# Autodesk Inventor assembly: Trunk
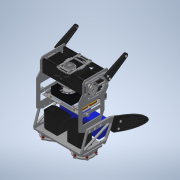
[picture p0: Inventor's stored thumbnail of the model, 180x180]
Saved by Autodesk Inventor 2020.4 (Build 244396000, 396)
## iProperties
Created: 2021-09-10
Part Number: Trunk
Document SubType Name: Assembly
Designer: Masato
Mass: 1616.91 g
Surface Area: 5782.28 cm^2
Volume: 882.028 cm^3
Density: 1.83317 g/cm^3
Author: Masato
## Documents named in this file (27)
- C:\Users\Masato\Documents\Inventor\CIT Brains_Inventor\OpenPlatform_ver3_0 - ve4_1 branch\UpperBody\Trunk\Trunk.iam
- C:\Users\Masato\Documents\Inventor\CIT Brains_Inventor\OpenPlatform_ver3_0 - ve4_1 branch\UpperBody\Trunk\Trunk_chest_horizontal_frame.ipt
- C:\Users\Masato\Documents\Inventor\CIT Brains_Inventor\OpenPlatform_ver3_0 - ve4_1 branch\UpperBody\Trunk\Trunk_chest_back_forth_frame.ipt
- C:\Users\Masato\Documents\Inventor\CIT Brains_Inventor\OpenPlatform_ver3_0 - ve4_1 branch\UpperBody\Trunk\Trunk_upper_flank_frame.ipt
- C:\Users\Masato\Documents\Inventor\CIT Brains_Inventor\OpenPlatform_ver3_0 - ve4_1 branch\UpperBody\Trunk\Trunk_shoulder_frame.ipt
- C:\Users\Masato\Documents\Inventor\CIT Brains_Inventor\OpenPlatform_ver3_0 - ve4_1 branch\UpperBody\Trunk\Trunk_handle_frame.ipt
- C:\Users\Masato\Documents\Inventor\CIT Brains_Inventor\OpenPlatform_ver3_0 - ve4_1 branch\Ready_Made\B3M11xx.ipt
- C:\Users\Masato\Documents\Inventor\CIT Brains_Inventor\OpenPlatform_ver3_0 - ve4_1 branch\Ready_Made\B3M10xx.ipt
- C:\Users\Masato\Documents\Inventor\CIT Brains_Inventor\OpenPlatform_ver3_0 - ve4_1 branch\UpperBody\Trunk\Trunk_shoulder_frame_MIR.ipt
- C:\Users\Masato\Documents\Inventor\CIT Brains_Inventor\OpenPlatform_ver3_0 - ve4_1 branch\UpperBody\Trunk\Trunk_lower_flank_frame.ipt
- C:\Users\Masato\Documents\Inventor\CIT Brains_Inventor\OpenPlatform_ver3_0 - ve4_1 branch\Ready_Made\Screw\SPNFL-BRN-M3-6.ipt
- C:\Users\Masato\Documents\Inventor\CIT Brains_Inventor\OpenPlatform_ver3_0 - ve4_1 branch\Ready_Made\Screw\M2_6-15.ipt
- C:\Users\Masato\Documents\Inventor\CIT Brains_Inventor\OpenPlatform_ver3_0 - ve4_1 branch\Ready_Made\Screw\M3-8.ipt
- C:\Users\Masato\Documents\Inventor\CIT Brains_Inventor\OpenPlatform_ver3_0 - ve4_1 branch\Ready_Made\Screw\M3-6.ipt
- C:\Users\Masato\Documents\Inventor\CIT Brains_Inventor\OpenPlatform_ver3_0 - ve4_1 branch\Ready_Made\Screw\M2_6-20.ipt
- C:\Users\Masato\Documents\Inventor\CIT Brains_Inventor\OpenPlatform_ver3_0 - ve4_1 branch\Ready_Made\BRU-309S.ipt
- C:\Users\Masato\Documents\Inventor\CIT Brains_Inventor\OpenPlatform_ver3_0 - ve4_1 branch\Ready_Made\UUW-0312-10BH.ipt
- C:\Users\Masato\Documents\Inventor\CIT Brains_Inventor\OpenPlatform_ver3_0 - ve4_1 branch\Ready_Made\ARU-306S.ipt
- C:\Users\Masato\Documents\Inventor\CIT Brains_Inventor\OpenPlatform_ver3_0 - ve4_1 branch\Ready_Made\SF319.ipt
- C:\Users\Masato\Documents\Inventor\CIT Brains_Inventor\OpenPlatform_ver3_0 - ve4_1 branch\UpperBody\Trunk\Trunk_back_bumper.ipt
- C:\Users\Masato\Documents\Inventor\CIT Brains_Inventor\OpenPlatform_ver3_0 - ve4_1 branch\Ready_Made\Screw\ClampHorn_Screw.ipt
- C:\Users\Masato\Documents\Inventor\CIT Brains_Inventor\OpenPlatform_ver3_0 - ve4_1 branch\Ready_Made\ClampHorn.ipt
- C:\Users\Masato\Documents\Inventor\CIT Brains_Inventor\OpenPlatform_ver3_0 - ve4_1 branch\Ready_Made\Jetson_Xavier_NX_DevKit_without_Wi-FiAntennas\Jetson_Xavier_NX_DevKit.ipt
- C:\Users\Masato\Documents\Inventor\CIT Brains_Inventor\OpenPlatform_ver3_0 - ve4_1 branch\Ready_Made\HP-G570-2600S3.ipt
- C:\Users\Masato\Documents\Inventor\CIT Brains_Inventor\OpenPlatform_ver3_0 - ve4_1 branch\UpperBody\Trunk\Trunk_lower_waisit_frame_.ipt
- C:\Users\Masato\Documents\Inventor\CIT Brains_Inventor\OpenPlatform_ver3_0 - ve4_1 branch\UpperBody\Trunk\CrossRollerBearing\BearingUnit.iam
- ClampHorn.ipt
## Components (98 placed, 25 different names)
1. Trunk_chest_horizontal_frame:1 — 挿入:172, 挿入:173, 挿入:174, 挿入:175, 挿入:177, 挿入:179, 挿入:255, 挿入:256, 挿入:261, 挿入:262, 挿入:347, 挿入:348
2. Trunk_chest_horizontal_frame:2 — 挿入:181, 挿入:182, 挿入:184, 挿入:185, 挿入:186, 挿入:187, 挿入:257, 挿入:258, 挿入:337, 挿入:338, 挿入:465, 挿入:466, 挿入:664, 挿入:665
3. Trunk_chest_back_forth_frame:1 — 挿入:115, 挿入:116, 挿入:117, 挿入:118, 挿入:172, 挿入:173, 挿入:181, 挿入:182
4. Trunk_chest_back_forth_frame:2 — 挿入:154, 挿入:155, 挿入:156, 挿入:157, 挿入:174, 挿入:175, 挿入:185, 挿入:187
5. Trunk_lower_flank_frame:1 — 挿入:501, 挿入:502, 挿入:668, 挿入:669, 挿入:692, 角度:3
6. Trunk_lower_flank_frame:2 — 挿入:499, 挿入:500, 挿入:666, 挿入:667, 挿入:691, メイト:3, メイト:4, 角度:2
7. Trunk_upper_flank_frame:1 — 挿入:115, 挿入:116, 挿入:156, 挿入:157, 挿入:226, 挿入:251, 挿入:252, 挿入:349, 挿入:350, フラッシュ:2, メイト:4, 挿入:699, 挿入:700, メイト:3
8. Trunk_upper_flank_frame:2 — 挿入:117, 挿入:118, 挿入:154, 挿入:155, 挿入:227, 挿入:253, 挿入:254, 挿入:351, 挿入:352, 挿入:697, 挿入:698
9. Trunk_shoulder_frame:1 — 挿入:559, 挿入:560, 挿入:561, 挿入:562, 挿入:563, 挿入:564, 挿入:565, 挿入:566, 挿入:571, 挿入:572, 挿入:573, 挿入:574, 挿入:699, 挿入:700
10. Trunk_shoulder_frame_MIR:1 — 挿入:581, 挿入:582, 挿入:583, 挿入:584, 挿入:587, 挿入:588, 挿入:589, 挿入:590, 挿入:591, 挿入:592, 挿入:593, 挿入:594, 挿入:595, 挿入:596, 挿入:697, 挿入:698
11. Trunk_handle_frame:1 — 挿入:263, 挿入:264, 挿入:267, 挿入:575, 挿入:576
12. Trunk_handle_frame:2 — 挿入:265, 挿入:266, 挿入:268, 挿入:597, 挿入:598
13. B3M11xx:3 — 挿入:177, 挿入:179, 挿入:184, 挿入:186, 挿入:681, 挿入:686
14. B3M10xx:4 — 挿入:559, 挿入:560, 挿入:561, 挿入:562, 挿入:679, 挿入:684
15. B3M10xx:5 — 挿入:581, 挿入:582, 挿入:583, 挿入:584, 挿入:680, 挿入:685
16. SPNFL-BRN-M3-6:1 — 挿入:226
17. SPNFL-BRN-M3-6:2 — 挿入:227
18. M3-6:1 — 挿入:251
19. M3-6:2 — 挿入:252
20. M3-6:3 — 挿入:254
21. M3-6:4 — 挿入:253
22. M3-6:5 — 挿入:256
23. M3-6:6 — 挿入:255
24. M3-6:7 — 挿入:258
25. M3-6:8 — 挿入:257
26. M2_6-15:11 — 挿入:261
27. M2_6-15:12 — 挿入:262
28. M3-6:9 — 挿入:263
29. M3-6:10 — 挿入:264
30. M3-6:11 — 挿入:266
31. M3-6:12 — 挿入:265
32. M3-8:11 — 挿入:267
33. M3-8:12 — 挿入:268
34. M2_6-15:13 — 挿入:564
35. M2_6-15:14 — 挿入:563
36. M2_6-15:15 — 挿入:566
37. M2_6-15:16 — 挿入:565
38. M2_6-15:17 — 挿入:591
39. M2_6-15:18 — 挿入:592
40. M2_6-15:19 — 挿入:589
41. M2_6-15:20 — 挿入:590
42. M3-6:19 — 挿入:587
43. M3-6:20 — 挿入:588
44. M2_6-20:9 — 挿入:465
45. M2_6-20:10 — 挿入:466
46. M2_6-20:11 — 挿入:337
47. M2_6-20:12 — 挿入:338
48. M3-6:29 — 挿入:347
49. M3-6:30 — 挿入:348
50. M3-6:31 — 挿入:349
51. M3-6:32 — 挿入:350
52. M3-6:33 — 挿入:351
53. M3-6:34 — 挿入:352
54. BRU-309S:9 — 挿入:497, 挿入:503
55. BRU-309S:10 — 挿入:498, 挿入:504
56. BRU-309S:11 — 挿入:496, 挿入:506
57. BRU-309S:12 — 挿入:495, 挿入:505
58. UUW-0312-10BH:1 — 挿入:495, 挿入:507
59. UUW-0312-10BH:2 — 挿入:496, 挿入:508
60. UUW-0312-10BH:3 — 挿入:497, 挿入:509
61. UUW-0312-10BH:4 — 挿入:498, 挿入:510
62. UUW-0312-10BH:5 — 挿入:499, 挿入:505, 挿入:672
63. UUW-0312-10BH:6 — 挿入:500, 挿入:506, 挿入:673
64. UUW-0312-10BH:7 — 挿入:501, 挿入:503, 挿入:674
65. UUW-0312-10BH:8 — 挿入:502, 挿入:504, 挿入:675
66. M3-6:43 — 挿入:507
67. M3-6:44 — 挿入:508
68. M3-6:45 — 挿入:510
69. M3-6:46 — 挿入:509
70. ARU-306S:1 — 挿入:571, 挿入:576
71. ARU-306S:2 — 挿入:572, 挿入:575
72. M3-6:55 — 挿入:573
73. M3-6:56 — 挿入:574
74. M3-6:57 — 挿入:593
75. M3-6:58 — 挿入:594
76. ARU-306S:3 — 挿入:595, 挿入:597
77. ARU-306S:4 — 挿入:596, 挿入:598
78. M3-6:59 — 挿入:664
79. M3-6:60 — 挿入:665
80. SF319:1 — 挿入:666
81. SF319:2 — 挿入:667
82. SF319:3 — 挿入:668
83. SF319:4 — 挿入:669
84. Trunk_back_bumper:1 — 挿入:672, 挿入:673
85. Trunk_back_bumper:2 — 挿入:674, 挿入:675
86. ClampHorn_Screw:3 — 挿入:684
87. ClampHorn_Screw:4 — 挿入:685
88. ClampHorn_Screw:5 — 挿入:686
89. ClampHorn:3 — 挿入:679
90. ClampHorn:4 — 挿入:680
91. ClampHorn:5 — 挿入:681
92. B3M11xx:1 — 挿入:689, 挿入:690
93. B3M11xx:2 — 挿入:687, 挿入:688
94. Jetson_Xavier_NX_DevKit:1
95. HP-G570-2600S3:1
96. Trunk_lower_waisit_frame_:1 — フラッシュ:1, 挿入:687, 挿入:688, 挿入:689, 挿入:690, 挿入:691, 挿入:692, フラッシュ:2, 角度:2, 角度:3, 挿入:693, 挿入:694, 挿入:695, 挿入:696, メイト:5
97. BearingUnit:1 [sub-assembly] — 挿入:694, 挿入:695
98. BearingUnit:2 [sub-assembly] — 挿入:693, 挿入:696
## Relationships (131: Insert 124, Mate 3, Flush 2, Angle 2)
- 挿入:115 [Insert]: Trunk_chest_back_forth_frame:1 ↔ Trunk_upper_flank_frame:1
- 挿入:116 [Insert]: Trunk_chest_back_forth_frame:1 ↔ Trunk_upper_flank_frame:1
- 挿入:117 [Insert]: Trunk_chest_back_forth_frame:1 ↔ Trunk_upper_flank_frame:2
- 挿入:118 [Insert]: Trunk_chest_back_forth_frame:1 ↔ Trunk_upper_flank_frame:2
- 挿入:154 [Insert]: Trunk_chest_back_forth_frame:2 ↔ Trunk_upper_flank_frame:2
- 挿入:155 [Insert]: Trunk_chest_back_forth_frame:2 ↔ Trunk_upper_flank_frame:2
- 挿入:156 [Insert]: Trunk_chest_back_forth_frame:2 ↔ Trunk_upper_flank_frame:1
- 挿入:157 [Insert]: Trunk_chest_back_forth_frame:2 ↔ Trunk_upper_flank_frame:1
- 挿入:172 [Insert]: Trunk_chest_horizontal_frame:1 ↔ Trunk_chest_back_forth_frame:1
- 挿入:173 [Insert]: Trunk_chest_horizontal_frame:1 ↔ Trunk_chest_back_forth_frame:1
- 挿入:174 [Insert]: Trunk_chest_horizontal_frame:1 ↔ Trunk_chest_back_forth_frame:2
- 挿入:175 [Insert]: Trunk_chest_horizontal_frame:1 ↔ Trunk_chest_back_forth_frame:2
- 挿入:177 [Insert]: Trunk_chest_horizontal_frame:1 ↔ B3M11xx:3
- 挿入:179 [Insert]: Trunk_chest_horizontal_frame:1 ↔ B3M11xx:3
- 挿入:181 [Insert]: Trunk_chest_horizontal_frame:2 ↔ Trunk_chest_back_forth_frame:1
- 挿入:182 [Insert]: Trunk_chest_horizontal_frame:2 ↔ Trunk_chest_back_forth_frame:1
- 挿入:184 [Insert]: Trunk_chest_horizontal_frame:2 ↔ B3M11xx:3
- 挿入:185 [Insert]: Trunk_chest_horizontal_frame:2 ↔ Trunk_chest_back_forth_frame:2
- 挿入:186 [Insert]: Trunk_chest_horizontal_frame:2 ↔ B3M11xx:3
- 挿入:187 [Insert]: Trunk_chest_horizontal_frame:2 ↔ Trunk_chest_back_forth_frame:2
- 挿入:226 [Insert]: Trunk_upper_flank_frame:1 ↔ SPNFL-BRN-M3-6:1
- 挿入:227 [Insert]: Trunk_upper_flank_frame:2 ↔ SPNFL-BRN-M3-6:2
- 挿入:251 [Insert]: Trunk_upper_flank_frame:1 ↔ M3-6:1
- 挿入:252 [Insert]: Trunk_upper_flank_frame:1 ↔ M3-6:2
- 挿入:253 [Insert]: Trunk_upper_flank_frame:2 ↔ M3-6:4
- 挿入:254 [Insert]: Trunk_upper_flank_frame:2 ↔ M3-6:3
- 挿入:255 [Insert]: Trunk_chest_horizontal_frame:1 ↔ M3-6:6
- 挿入:256 [Insert]: Trunk_chest_horizontal_frame:1 ↔ M3-6:5
- 挿入:257 [Insert]: Trunk_chest_horizontal_frame:2 ↔ M3-6:8
- 挿入:258 [Insert]: Trunk_chest_horizontal_frame:2 ↔ M3-6:7
- 挿入:261 [Insert]: Trunk_chest_horizontal_frame:1 ↔ M2_6-15:11
- 挿入:262 [Insert]: Trunk_chest_horizontal_frame:1 ↔ M2_6-15:12
- 挿入:263 [Insert]: Trunk_handle_frame:1 ↔ M3-6:9
- 挿入:264 [Insert]: Trunk_handle_frame:1 ↔ M3-6:10
- 挿入:265 [Insert]: Trunk_handle_frame:2 ↔ M3-6:12
- 挿入:266 [Insert]: Trunk_handle_frame:2 ↔ M3-6:11
- 挿入:267 [Insert]: Trunk_handle_frame:1 ↔ M3-8:11
- 挿入:268 [Insert]: Trunk_handle_frame:2 ↔ M3-8:12
- 挿入:337 [Insert]: Trunk_chest_horizontal_frame:2 ↔ M2_6-20:11
- 挿入:338 [Insert]: Trunk_chest_horizontal_frame:2 ↔ M2_6-20:12
- 挿入:347 [Insert]: Trunk_chest_horizontal_frame:1 ↔ M3-6:29
- 挿入:348 [Insert]: Trunk_chest_horizontal_frame:1 ↔ M3-6:30
- 挿入:349 [Insert]: Trunk_upper_flank_frame:1 ↔ M3-6:31
- 挿入:350 [Insert]: Trunk_upper_flank_frame:1 ↔ M3-6:32
- 挿入:351 [Insert]: Trunk_upper_flank_frame:2 ↔ M3-6:33
- 挿入:352 [Insert]: Trunk_upper_flank_frame:2 ↔ M3-6:34
- 挿入:465 [Insert]: Trunk_chest_horizontal_frame:2 ↔ M2_6-20:9
- 挿入:466 [Insert]: Trunk_chest_horizontal_frame:2 ↔ M2_6-20:10
- 挿入:495 [Insert]: BRU-309S:12 ↔ UUW-0312-10BH:1
- 挿入:496 [Insert]: BRU-309S:11 ↔ UUW-0312-10BH:2
- 挿入:497 [Insert]: BRU-309S:9 ↔ UUW-0312-10BH:3
- 挿入:498 [Insert]: BRU-309S:10 ↔ UUW-0312-10BH:4
- 挿入:499 [Insert]: Trunk_lower_flank_frame:2 ↔ UUW-0312-10BH:5
- 挿入:500 [Insert]: Trunk_lower_flank_frame:2 ↔ UUW-0312-10BH:6
- 挿入:501 [Insert]: Trunk_lower_flank_frame:1 ↔ UUW-0312-10BH:7
- 挿入:502 [Insert]: Trunk_lower_flank_frame:1 ↔ UUW-0312-10BH:8
- 挿入:503 [Insert]: BRU-309S:9 ↔ UUW-0312-10BH:7
- 挿入:504 [Insert]: BRU-309S:10 ↔ UUW-0312-10BH:8
- 挿入:505 [Insert]: BRU-309S:12 ↔ UUW-0312-10BH:5
- 挿入:506 [Insert]: BRU-309S:11 ↔ UUW-0312-10BH:6
- 挿入:507 [Insert]: UUW-0312-10BH:1 ↔ M3-6:43
- 挿入:508 [Insert]: UUW-0312-10BH:2 ↔ M3-6:44
- 挿入:509 [Insert]: UUW-0312-10BH:3 ↔ M3-6:46
- 挿入:510 [Insert]: UUW-0312-10BH:4 ↔ M3-6:45
- 挿入:559 [Insert]: Trunk_shoulder_frame:1 ↔ B3M10xx:4
- 挿入:560 [Insert]: Trunk_shoulder_frame:1 ↔ B3M10xx:4
- 挿入:561 [Insert]: Trunk_shoulder_frame:1 ↔ B3M10xx:4
- 挿入:562 [Insert]: Trunk_shoulder_frame:1 ↔ B3M10xx:4
- 挿入:563 [Insert]: Trunk_shoulder_frame:1 ↔ M2_6-15:14
- 挿入:564 [Insert]: Trunk_shoulder_frame:1 ↔ M2_6-15:13
- 挿入:565 [Insert]: Trunk_shoulder_frame:1 ↔ M2_6-15:16
- 挿入:566 [Insert]: Trunk_shoulder_frame:1 ↔ M2_6-15:15
- 挿入:571 [Insert]: Trunk_shoulder_frame:1 ↔ ARU-306S:1
- 挿入:572 [Insert]: Trunk_shoulder_frame:1 ↔ ARU-306S:2
- 挿入:573 [Insert]: Trunk_shoulder_frame:1 ↔ M3-6:55
- 挿入:574 [Insert]: Trunk_shoulder_frame:1 ↔ M3-6:56
- 挿入:575 [Insert]: Trunk_handle_frame:1 ↔ ARU-306S:2
- 挿入:576 [Insert]: Trunk_handle_frame:1 ↔ ARU-306S:1
- 挿入:581 [Insert]: Trunk_shoulder_frame_MIR:1 ↔ B3M10xx:5
- 挿入:582 [Insert]: Trunk_shoulder_frame_MIR:1 ↔ B3M10xx:5
- 挿入:583 [Insert]: Trunk_shoulder_frame_MIR:1 ↔ B3M10xx:5
- 挿入:584 [Insert]: Trunk_shoulder_frame_MIR:1 ↔ B3M10xx:5
- 挿入:587 [Insert]: Trunk_shoulder_frame_MIR:1 ↔ M3-6:19
- 挿入:588 [Insert]: Trunk_shoulder_frame_MIR:1 ↔ M3-6:20
- 挿入:589 [Insert]: Trunk_shoulder_frame_MIR:1 ↔ M2_6-15:19
- 挿入:590 [Insert]: Trunk_shoulder_frame_MIR:1 ↔ M2_6-15:20
- 挿入:591 [Insert]: Trunk_shoulder_frame_MIR:1 ↔ M2_6-15:17
- 挿入:592 [Insert]: Trunk_shoulder_frame_MIR:1 ↔ M2_6-15:18
- 挿入:593 [Insert]: Trunk_shoulder_frame_MIR:1 ↔ M3-6:57
- 挿入:594 [Insert]: Trunk_shoulder_frame_MIR:1 ↔ M3-6:58
- 挿入:595 [Insert]: Trunk_shoulder_frame_MIR:1 ↔ ARU-306S:3
- 挿入:596 [Insert]: Trunk_shoulder_frame_MIR:1 ↔ ARU-306S:4
- 挿入:597 [Insert]: Trunk_handle_frame:2 ↔ ARU-306S:3
- 挿入:598 [Insert]: Trunk_handle_frame:2 ↔ ARU-306S:4
- 挿入:664 [Insert]: Trunk_chest_horizontal_frame:2 ↔ M3-6:59
- 挿入:665 [Insert]: Trunk_chest_horizontal_frame:2 ↔ M3-6:60
- 挿入:666 [Insert]: Trunk_lower_flank_frame:2 ↔ SF319:1
- 挿入:667 [Insert]: Trunk_lower_flank_frame:2 ↔ SF319:2
- 挿入:668 [Insert]: Trunk_lower_flank_frame:1 ↔ SF319:3
- 挿入:669 [Insert]: Trunk_lower_flank_frame:1 ↔ SF319:4
- 挿入:672 [Insert]: UUW-0312-10BH:5 ↔ Trunk_back_bumper:1
- 挿入:673 [Insert]: UUW-0312-10BH:6 ↔ Trunk_back_bumper:1
- 挿入:674 [Insert]: UUW-0312-10BH:7 ↔ Trunk_back_bumper:2
- 挿入:675 [Insert]: UUW-0312-10BH:8 ↔ Trunk_back_bumper:2
- 挿入:679 [Insert]: B3M10xx:4 ↔ ClampHorn:3
- 挿入:680 [Insert]: B3M10xx:5 ↔ ClampHorn:4
- 挿入:681 [Insert]: B3M11xx:3 ↔ ClampHorn:5
- 挿入:684 [Insert]: B3M10xx:4 ↔ ClampHorn_Screw:3
- 挿入:685 [Insert]: B3M10xx:5 ↔ ClampHorn_Screw:4
- 挿入:686 [Insert]: B3M11xx:3 ↔ ClampHorn_Screw:5
- フラッシュ:1 [Flush]: Trunk_lower_waisit_frame_:1
- 挿入:687 [Insert]: B3M11xx:2 ↔ Trunk_lower_waisit_frame_:1
- 挿入:688 [Insert]: B3M11xx:2 ↔ Trunk_lower_waisit_frame_:1
- 挿入:689 [Insert]: B3M11xx:1 ↔ Trunk_lower_waisit_frame_:1
- 挿入:690 [Insert]: B3M11xx:1 ↔ Trunk_lower_waisit_frame_:1
- 挿入:691 [Insert]: Trunk_lower_flank_frame:2 ↔ Trunk_lower_waisit_frame_:1
- 挿入:692 [Insert]: Trunk_lower_flank_frame:1 ↔ Trunk_lower_waisit_frame_:1
- フラッシュ:2 [Flush]: Trunk_upper_flank_frame:1 ↔ Trunk_lower_waisit_frame_:1
- メイト:3 [Mate] (3 mm): Trunk_lower_flank_frame:2 ↔ Trunk_upper_flank_frame:1
- メイト:4 [Mate] (-10 mm): Trunk_lower_flank_frame:2 ↔ Trunk_upper_flank_frame:1
- 角度:2 [Angle] (0 deg): Trunk_lower_flank_frame:2 ↔ Trunk_lower_waisit_frame_:1
- 角度:3 [Angle] (0 deg): Trunk_lower_flank_frame:1 ↔ Trunk_lower_waisit_frame_:1
- 挿入:693 [Insert]: Trunk_lower_waisit_frame_:1 ↔ BearingUnit:2
- 挿入:694 [Insert]: Trunk_lower_waisit_frame_:1 ↔ BearingUnit:1
- 挿入:695 [Insert]: Trunk_lower_waisit_frame_:1 ↔ BearingUnit:1
- 挿入:696 [Insert]: Trunk_lower_waisit_frame_:1 ↔ BearingUnit:2
- 挿入:697 [Insert]: Trunk_upper_flank_frame:2 ↔ Trunk_shoulder_frame_MIR:1
- 挿入:698 [Insert]: Trunk_upper_flank_frame:2 ↔ Trunk_shoulder_frame_MIR:1
- メイト:5 [Mate]: Trunk_lower_waisit_frame_:1
- 挿入:699 [Insert]: Trunk_upper_flank_frame:1 ↔ Trunk_shoulder_frame:1
- 挿入:700 [Insert]: Trunk_upper_flank_frame:1 ↔ Trunk_shoulder_frame:1
